# Autodesk Inventor assembly: beercart assembly - mekatronik
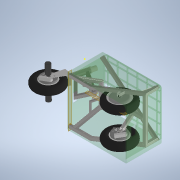
[picture p0: Inventor's stored thumbnail of the model, 180x180]
Saved by Autodesk Inventor 2022.2 (Build 262287010, 287A)
## iProperties
_SolveAssemblyDoc: Frame Generator Solve Assembly
_Version: 15.0.0
Created: 2022-03-11
Part Number: beercart assembly - mekatronik
Document SubType Name: Assembly
Designer: foriw
Mass: 9959.72 g
Surface Area: 13437.1 cm^2
Volume: 7103.99 cm^3
Density: 1.40199 g/cm^3
Author: foriw
## Documents named in this file (15)
- C:\Users\Finn Oriwohl\Documents\htx\1g g\BeerCart-CAD-Inventor\Workspaces\Workspace\beercart assembly - mekatronik.iam
- C:\Users\Finn Oriwohl\Documents\htx\1g g\BeerCart-CAD-Inventor\Workspaces\Workspace\beercart- framwork - baseSketch.ipt
- C:\Users\Finn Oriwohl\Documents\htx\1g g\BeerCart-CAD-Inventor\Workspaces\Workspace\beercart assembly - mekatronik\Frame\Frame 1647030135921.iam
- C:\Users\Finn Oriwohl\Documents\htx\1g g\BeerCart-CAD-Inventor\Workspaces\Workspace\beer crate.ipt
- C:\Users\Finn Oriwohl\Documents\htx\1g g\BeerCart-CAD-Inventor\Workspaces\Workspace\Mekatronik-beerCart\frontwheel frame.ipt
- C:\Users\Finn Oriwohl\Documents\htx\1g g\BeerCart-CAD-Inventor\Workspaces\Workspace\motor at24v_MIR.ipt
- C:\Users\Finn Oriwohl\Documents\htx\1g g\BeerCart-CAD-Inventor\Workspaces\Workspace\FreeBackWheel.ipt
- C:\Users\Finn Oriwohl\Documents\htx\1g g\BeerCart-CAD-Inventor\Libraries\Content Center Files\en-US\ANSI B18.2.4.4M\ANSI B18.2.4.4M - M8 x 1,25.ipt
- C:\Users\Finn Oriwohl\Documents\htx\1g g\BeerCart-CAD-Inventor\Libraries\Content Center Files\en-US\DIN 6923\DIN 6923 - M8 x 1.25.ipt
- C:\Users\Finn Oriwohl\Documents\htx\1g g\BeerCart-CAD-Inventor\Workspaces\Workspace\rotating axel.ipt
- C:\Users\Finn Oriwohl\Documents\htx\1g g\BeerCart-CAD-Inventor\Workspaces\Workspace\beercart assembly - mekatronik\AIP\FEA\dxkkndp9c.fins
- C:\Users\Finn Oriwohl\Documents\htx\1g g\BeerCart-CAD-Inventor\Workspaces\Workspace\beercart assembly - mekatronik\AIP\FEA\dxkkndp9c.fsat
- C:\Users\Finn Oriwohl\Documents\htx\1g g\BeerCart-CAD-Inventor\Workspaces\Workspace\beercart assembly - mekatronik\AIP\FEA\dxkkndp9c.ftes
- C:\Users\Finn Oriwohl\Documents\htx\1g g\BeerCart-CAD-Inventor\Workspaces\Workspace\beercart assembly - mekatronik\AIP\FEA\dxkkndpa8.fwiz
- C:\Users\Finn Oriwohl\Documents\htx\1g g\BeerCart-CAD-Inventor\Workspaces\Workspace\beercart assembly - mekatronik\AIP\FEA\dxkkndpfk.fmsh
## Components (10 placed, 9 different names)
1. beercart- framwork - baseSketch:1
2. Frame 1647030135921:1 [sub-assembly] — Flush:3, Insert:2, Insert:3, Mate:2, Insert:4, Mate:3, Insert:5, Angle:1, Insert:6, Insert:7, Mate:5, Mate:6
3. beer crate:1 — Flush:2, Flush:3
4. frontwheel frame:1 — Flush:4, Mate:4
5. motor at24v_MIR:1 — Insert:2, Insert:3, Mate:1, Insert:5, Angle:1
6. FreeBackWheel:1 — Mate:1, Mate:2, Mate:3
7. Metric Hex Flange Nuts - Metric M8 x 1,25:1 — Insert:4
8. DIN 6923 M8:1 — Insert:6
9. DIN 6923 M8:2 — Insert:7
10. rotating axel:1 — Mate:4, Mate:5, Mate:6
## Relationships (17: Insert 7, Mate 6, Flush 3, Angle 1)
- Flush:2: beer crate:1
- Flush:3: Frame 1647030135921:1 ↔ beer crate:1
- [Insert]: Frame 1647030135921:1 ↔ motor at24v_MIR:1
- Insert:2: Frame 1647030135921:1 ↔ motor at24v_MIR:1
- Insert:3: Frame 1647030135921:1 ↔ motor at24v_MIR:1
- Mate:1: motor at24v_MIR:1 ↔ FreeBackWheel:1
- Mate:2 (0.5 mm): Frame 1647030135921:1 ↔ FreeBackWheel:1
- Insert:4: Frame 1647030135921:1 ↔ Metric Hex Flange Nuts - Metric M8 x 1,25:1
- Mate:3 (0.5 mm): Frame 1647030135921:1 ↔ FreeBackWheel:1
- Insert:5: Frame 1647030135921:1 ↔ motor at24v_MIR:1
- Angle:1 (0 deg): Frame 1647030135921:1 ↔ motor at24v_MIR:1
- Insert:6: Frame 1647030135921:1 ↔ DIN 6923 M8:1
- Flush:4: frontwheel frame:1
- Insert:7: Frame 1647030135921:1 ↔ DIN 6923 M8:2
- Mate:4: frontwheel frame:1 ↔ rotating axel:1
- Mate:5: Frame 1647030135921:1 ↔ rotating axel:1
- Mate:6: Frame 1647030135921:1 ↔ rotating axel:1
## Named parameters: sa_0 = 0, sa_1 = -148100, sa_2 = 0
note: some values were not read from the file. Shown as the stored number, unit unknown: "sa_0", "sa_1", "sa_2".
